# Autodesk Inventor assembly: 3D_Drucker_v02
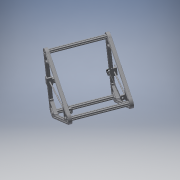
[picture p0: Inventor's stored thumbnail of the model, 180x180]
Saved by Autodesk Inventor 2019 (Build 230136000, 136)
## iProperties
Created: 2018-08-19
Part Number: 3D_Drucker_v02
Document SubType Name: Assembly
Designer: Julia
Author: Julia
## Documents named in this file (3)
- C:\Users\Julia\Documents\Inventor\3d_Drucker_v04_Single_Y_Fuehrung\3D_Drucker_v03.iam
- C:\Users\Julia\Documents\Inventor\3d_Drucker_v04_Single_Y_Fuehrung\Rahmen.iam
- C:\Users\Julia\Documents\Inventor\3d_Drucker_v04_Single_Y_Fuehrung\Y_Führung.iam
## Components (3 placed, 2 different names)
1. Rahmen:1 [sub-assembly] — Mate:23, Mate:24, Mate:25
2. Y_Führung:1 [sub-assembly] — Mate:23, Mate:24, Mate:25
3. Y_Führung:2 [sub-assembly]
## Relationships (3: Mate 3)
- Mate:23: Rahmen:1 ↔ Y_Führung:1
- Mate:24: Rahmen:1 ↔ Y_Führung:1
- Mate:25: Rahmen:1 ↔ Y_Führung:1
